# Autodesk Inventor assembly: KaszmirCały
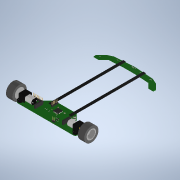
[picture p0: Inventor's stored thumbnail of the model, 180x180]
Saved by Autodesk Inventor 2021 (Build 250183000, 183)
## iProperties
Created: 2021-05-05
Part Number: KaszmirCały
Document SubType Name: Assembly
Designer: kriso
Author: kriso
## Documents named in this file (7)
- C:\Users\kriso\Documents\1. STUDIA\6 semestr\RobotyMobilne\Kaszmir_Inventor\KaszmirCały.iam
- C:\Users\kriso\Documents\1. STUDIA\6 semestr\RobotyMobilne\Kaszmir\Kaszmir\Kaszmir.iam
- C:\Users\kriso\Documents\1. STUDIA\6 semestr\RobotyMobilne\Kaszmir\Kaszmir\KaszmirSensors\KaszmirSensors.iam
- C:\Users\kriso\Documents\1. STUDIA\6 semestr\RobotyMobilne\Kaszmir_Inventor\pololu-2218-micro-metal-gearmotor-with-extended-motor-shaft-1.snapshot.1\Pololu #2218 Micro Metal Gearmotor HP.ipt
- C:\Users\kriso\Documents\1. STUDIA\6 semestr\RobotyMobilne\Kaszmir\Kaszmir\KaszmirSensors\Bracket.ipt
- C:\Users\kriso\Documents\1. STUDIA\6 semestr\RobotyMobilne\Kaszmir_Inventor\listwa_weglowa.ipt
- C:\Users\kriso\Documents\1. STUDIA\6 semestr\RobotyMobilne\Kaszmir_Inventor\wheel-solarbotics-rw2i-internally-mounted-1.snapshot.4\STEP\koło_solarbotics.ipt
## Components (10 placed, 6 different names)
1. Kaszmir:1 [sub-assembly] — Równoległe:1, Zestawiające:1, Równoległe:2, Zestawiające:2, Równoległe:3, Zestawiające:3, Zestawiające:5, Równoległe:4, Zestawiające:6, Zestawiające:7, Zestawiające:9, Zestawiające:10, Zestawiające:11, Zestawiające:12, Zestawiające:13, Zestawiające:14
2. KaszmirSensors:1 [sub-assembly] — Równoległe:1, Zestawiające:15, Zestawiające:16
3. Pololu #2218 Micro Metal Gearmotor HP:1 — Zestawiające:7, Równoległe:5, Zestawiające:8, Zestawiające:18, Równoległe:7
4. Bracket:1 — Zestawiające:5, Równoległe:4, Zestawiające:6, Równoległe:5, Zestawiające:8
5. Bracket:2 — Zestawiające:2, Równoległe:3, Zestawiające:3, Zestawiające:4
6. Pololu #2218 Micro Metal Gearmotor HP:2 — Zestawiające:1, Równoległe:2, Zestawiające:4, Zestawiające:17, Równoległe:6
7. listwa_weglowa:1 — Zestawiające:9, Zestawiające:10, Zestawiające:11
8. listwa_weglowa:2 — Zestawiające:12, Zestawiające:13, Zestawiające:14, Zestawiające:15, Zestawiające:16
9. koło_solarbotics:1 — Zestawiające:18, Równoległe:7
10. koło_solarbotics:2 — Zestawiające:17, Równoległe:6
## Relationships (25: Mate 18, Flush 7)
- Równoległe:1 [Flush]: Kaszmir:1 ↔ KaszmirSensors:1
- Zestawiające:1 [Mate]: Kaszmir:1 ↔ Pololu #2218 Micro Metal Gearmotor HP:2
- Równoległe:2 [Flush]: Kaszmir:1 ↔ Pololu #2218 Micro Metal Gearmotor HP:2
- Zestawiające:2 [Mate]: Kaszmir:1 ↔ Bracket:2
- Równoległe:3 [Flush]: Kaszmir:1 ↔ Bracket:2
- Zestawiające:3 [Mate]: Kaszmir:1 ↔ Bracket:2
- Zestawiające:4 [Mate]: Bracket:2 ↔ Pololu #2218 Micro Metal Gearmotor HP:2
- Zestawiające:5 [Mate]: Kaszmir:1 ↔ Bracket:1
- Równoległe:4 [Flush]: Kaszmir:1 ↔ Bracket:1
- Zestawiające:6 [Mate]: Kaszmir:1 ↔ Bracket:1
- Zestawiające:7 [Mate]: Kaszmir:1 ↔ Pololu #2218 Micro Metal Gearmotor HP:1
- Równoległe:5 [Flush]: Pololu #2218 Micro Metal Gearmotor HP:1 ↔ Bracket:1
- Zestawiające:8 [Mate]: Pololu #2218 Micro Metal Gearmotor HP:1 ↔ Bracket:1
- Zestawiające:9 [Mate]: Kaszmir:1 ↔ listwa_weglowa:1
- Zestawiające:10 [Mate]: Kaszmir:1 ↔ listwa_weglowa:1
- Zestawiające:11 [Mate]: Kaszmir:1 ↔ listwa_weglowa:1
- Zestawiające:12 [Mate]: Kaszmir:1 ↔ listwa_weglowa:2
- Zestawiające:13 [Mate]: Kaszmir:1 ↔ listwa_weglowa:2
- Zestawiające:14 [Mate]: Kaszmir:1 ↔ listwa_weglowa:2
- Zestawiające:15 [Mate]: KaszmirSensors:1 ↔ listwa_weglowa:2
- Zestawiające:16 [Mate]: KaszmirSensors:1 ↔ listwa_weglowa:2
- Zestawiające:17 [Mate]: Pololu #2218 Micro Metal Gearmotor HP:2 ↔ koło_solarbotics:2
- Równoległe:6 [Flush]: Pololu #2218 Micro Metal Gearmotor HP:2 ↔ koło_solarbotics:2
- Zestawiające:18 [Mate]: Pololu #2218 Micro Metal Gearmotor HP:1 ↔ koło_solarbotics:1
- Równoległe:7 [Flush]: Pololu #2218 Micro Metal Gearmotor HP:1 ↔ koło_solarbotics:1
